# Autodesk Inventor assembly: Project spacing
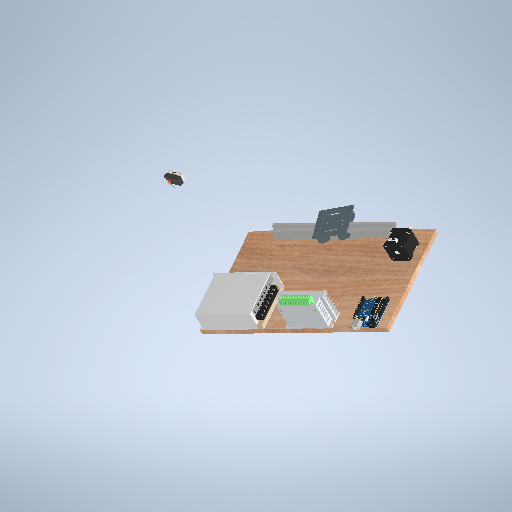
[picture p0: Inventor's stored thumbnail of the model, 512x512]
Saved by Autodesk Inventor 2025.1 (Build 291241000, 241)
## iProperties
Created: 2025-04-10
Part Number: Project spacing
Document SubType Name: Assembly
Designer: 6235654
Author: 6235654
## Documents named in this file (9)
- C:\Users\6235654\OneDrive - Vanier College\workshop 2\Project\Project spacing.iam
- C:\Users\6235654\OneDrive - Vanier College\workshop 2\extrusion\aluextrusion.ipt
- C:\Users\6235654\OneDrive - Vanier College\workshop 2\gantre\GANTREAssembly1.iam
- C:\Users\6235654\OneDrive - Vanier College\workshop 2\Assembly5.iam
- C:\Users\6235654\OneDrive - Vanier College\workshop 2\Project\TB6600.iam
- C:\Users\6235654\OneDrive - Vanier College\workshop 2\Nema 17 model v2\Nema 17 model v2\Nema 17 model v2.ipt
- C:\Users\6235654\OneDrive - Vanier College\workshop 2\Power Supply S-120-24 v1\Power Supply S-120-24 v1\Power Supply S-120-24 v1.ipt
- C:\Users\6235654\OneDrive - Vanier College\workshop 2\Arduino UNO\Arduino UNO\Arduino UNO\Arduino UNO.ipt
- C:\Users\6235654\OneDrive - Vanier College\workshop 2\Project\wood.ipt
## Components (8 placed, 8 different names)
1. aluextrusion:1 — Mate:4
2. GANTREAssembly1:1 [sub-assembly] — Mate:4
3. Assembly5:1 [sub-assembly]
4. TB6600:1 [sub-assembly] — Mate:2, Flush:4
5. Nema 17 model v2:1 — Mate:5
6. Power Supply S-120-24 v1:1 — Mate:1, Flush:3
7. Arduino UNO:1 — Mate:3, Flush:2
8. wood:1 — Mate:1, Mate:2, Mate:3, Flush:2, Mate:5, Flush:3, Flush:4
## Relationships (8: Mate 5, Flush 3)
- Mate:1: Power Supply S-120-24 v1:1 ↔ wood:1
- Mate:2: TB6600:1 ↔ wood:1
- Mate:3: Arduino UNO:1 ↔ wood:1
- Flush:2: Arduino UNO:1 ↔ wood:1
- Mate:4: aluextrusion:1 ↔ GANTREAssembly1:1
- Mate:5: Nema 17 model v2:1 ↔ wood:1
- Flush:3: Power Supply S-120-24 v1:1 ↔ wood:1
- Flush:4: TB6600:1 ↔ wood:1
